# Autodesk Inventor assembly: PCB
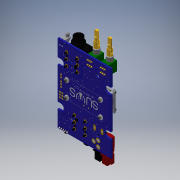
[picture p0: Inventor's stored thumbnail of the model, 180x180]
Saved by Autodesk Inventor 2016 (Build 200138000, 138)
## iProperties
Created: 2016-12-24
Part Number: PCB
Document SubType Name: Assembly
Designer: Tyler
Author: Tyler
## Documents named in this file (13)
- C:\Users\Tyler\Documents\Small Projects\Personal\morse-practice-oscillator\Mechanicial\Sounder\PCB.iam
- C:\Users\Tyler\Documents\Small Projects\Personal\morse-practice-oscillator\Mechanicial\Sounder\PCB.ipt
- C:\Users\Tyler\Documents\Small Projects\Personal\morse-practice-oscillator\Mechanicial\Sounder\Imported Components\3D+File+NRJ6HH\3D+File+NRJ6HH.ipt
- C:\Users\Tyler\Documents\Small Projects\Personal\morse-practice-oscillator\Mechanicial\Sounder\speaker.ipt
- C:\Users\Tyler\Documents\Small Projects\Personal\morse-practice-oscillator\Mechanicial\Sounder\speaker_standoff.ipt
- C:\Users\Tyler\Documents\Inventor\Content Center Files\R2016\en-US\ISO 7045  Z\ISO 7045 - M2 x 16 - 4.8 - Z - ISO.ipt
- C:\Users\Tyler\Documents\Inventor\Content Center Files\R2016\en-US\AS 1112 (2)\AS 1112 - M2  Type 5.ipt
- C:\Users\Tyler\Documents\Small Projects\Personal\morse-practice-oscillator\Mechanicial\Sounder\P082D.ipt
- C:\Users\Tyler\Documents\Small Projects\Personal\morse-practice-oscillator\Mechanicial\Sounder\Imported Components\PP 15-45 (Std)-02-08-STEP\PP 15-45 (Std)-02-08-STEP.ipt
- C:\Users\Tyler\Documents\Small Projects\Personal\morse-practice-oscillator\Mechanicial\Sounder\TE-1825232.ipt
- C:\Users\Tyler\Documents\Small Projects\Personal\morse-practice-oscillator\Mechanicial\Sounder\Multicomp-2118128.ipt
- C:\Users\Tyler\Documents\Small Projects\Personal\morse-practice-oscillator\Mechanicial\Sounder\pj-002b.ipt
- C:\Users\Tyler\Documents\Small Projects\Personal\morse-practice-oscillator\Mechanicial\Sounder\SLP3.ipt
## Components (24 placed, 12 different names)
1. PCB:1 — Flush:1, Mate:1, Mate:2, Flush:2, Mate:3, Mate:4, Insert:1, Insert:2, Insert:3, Insert:4, Insert:9, Insert:10, Insert:11, Insert:12, Mate:6, Mate:7, Flush:3, Flush:4, Mate:9, Angle:1, Mate:10, Mate:11, Mate:12, Mate:13, Mate:14, Mate:15, Mate:16, Flush:7, Flush:8, Mate:17, Flush:9, Mate:18, Mate:19, Mate:20, Mate:21, Mate:22, Flush:10, Mate:23
2. 3D+File+NRJ6HH:1 — Flush:1, Mate:1, Mate:10
3. 3D+File+NRJ6HH:2 — Mate:2, Flush:2, Mate:14
4. speaker:1 — Mate:3, Mate:4, Mate:5, Insert:5, Insert:6, Insert:7, Insert:8
5. speaker_standoff:1 — Insert:1
6. speaker_standoff:2 — Insert:2
7. speaker_standoff:3 — Insert:3, Mate:5
8. speaker_standoff:4 — Insert:4
9. ISO 7045 Z M2 x 16 - 4.8 - Z:1 — Insert:5
10. ISO 7045 Z M2 x 16 - 4.8 - Z:2 — Insert:6
11. ISO 7045 Z M2 x 16 - 4.8 - Z:3 — Insert:7
12. ISO 7045 Z M2 x 16 - 4.8 - Z:4 — Insert:8
13. AS 1112 (2) - Metric M2  Type 5:1 — Insert:9
14. AS 1112 (2) - Metric M2  Type 5:2 — Insert:10
15. AS 1112 (2) - Metric M2  Type 5:3 — Insert:11
16. AS 1112 (2) - Metric M2  Type 5:4 — Insert:12
17. P082D:1 — Mate:6, Flush:3, Mate:11
18. P082D:2 — Mate:7, Flush:4, Mate:12
19. PP 15-45 (Std)-02-08-STEP:1 — Mate:8, Flush:5, Flush:6, Mate:9, Angle:1
20. PP 15-45 (Std)-02-08-STEP:2 — Mate:8, Flush:5, Flush:6, Flush:7, Flush:8
21. TE-1825232:1 — Mate:13, Mate:15, Mate:16
22. Multicomp-2118128:1 — Mate:17, Flush:9, Mate:18
23. pj-002b:1 — Mate:19, Mate:20, Mate:21
24. SLP3:1 — Mate:22, Flush:10, Mate:23
## Relationships (46: Mate 23, Insert 12, Flush 10, Angle 1)
- Flush:1 (3.81 mm): PCB:1 ↔ 3D+File+NRJ6HH:1
- Mate:1: PCB:1 ↔ 3D+File+NRJ6HH:1
- Mate:2: PCB:1 ↔ 3D+File+NRJ6HH:2
- Flush:2 (3.81 mm): PCB:1 ↔ 3D+File+NRJ6HH:2
- Mate:3: PCB:1 ↔ speaker:1
- Mate:4: PCB:1 ↔ speaker:1
- Insert:1: PCB:1 ↔ speaker_standoff:1
- Insert:2: PCB:1 ↔ speaker_standoff:2
- Insert:3: PCB:1 ↔ speaker_standoff:3
- Insert:4: PCB:1 ↔ speaker_standoff:4
- Mate:5: speaker:1 ↔ speaker_standoff:3
- Insert:5: speaker:1 ↔ ISO 7045 Z M2 x 16 - 4.8 - Z:1
- Insert:6: speaker:1 ↔ ISO 7045 Z M2 x 16 - 4.8 - Z:2
- Insert:7: speaker:1 ↔ ISO 7045 Z M2 x 16 - 4.8 - Z:3
- Insert:8: speaker:1 ↔ ISO 7045 Z M2 x 16 - 4.8 - Z:4
- Insert:9: PCB:1 ↔ AS 1112 (2) - Metric M2  Type 5:1
- Insert:10: PCB:1 ↔ AS 1112 (2) - Metric M2  Type 5:2
- Insert:11: PCB:1 ↔ AS 1112 (2) - Metric M2  Type 5:3
- Insert:12: PCB:1 ↔ AS 1112 (2) - Metric M2  Type 5:4
- Mate:6: PCB:1 ↔ P082D:1
- Mate:7: PCB:1 ↔ P082D:2
- Flush:3: PCB:1 ↔ P082D:1
- Flush:4: PCB:1 ↔ P082D:2
- Mate:8: PP 15-45 (Std)-02-08-STEP:1 ↔ PP 15-45 (Std)-02-08-STEP:2
- Flush:5: PP 15-45 (Std)-02-08-STEP:1 ↔ PP 15-45 (Std)-02-08-STEP:2
- Flush:6: PP 15-45 (Std)-02-08-STEP:1 ↔ PP 15-45 (Std)-02-08-STEP:2
- Mate:9: PCB:1 ↔ PP 15-45 (Std)-02-08-STEP:1
- Angle:1 (180 deg): PCB:1 ↔ PP 15-45 (Std)-02-08-STEP:1
- Mate:10 (-13.97 mm): PCB:1 ↔ 3D+File+NRJ6HH:1
- Mate:11 (-34.29 mm): PCB:1 ↔ P082D:1
- Mate:12 (-48.26 mm): PCB:1 ↔ P082D:2
- Mate:13: PCB:1 ↔ TE-1825232:1
- Mate:14 (-25.4 mm): PCB:1 ↔ 3D+File+NRJ6HH:2
- Mate:15 (-6.35 mm): PCB:1 ↔ TE-1825232:1
- Mate:16 (-1.38 mm): PCB:1 ↔ TE-1825232:1
- Flush:7 (43.18 mm): PCB:1 ↔ PP 15-45 (Std)-02-08-STEP:2
- Flush:8 (69.85 mm): PCB:1 ↔ PP 15-45 (Std)-02-08-STEP:2
- Mate:17: PCB:1 ↔ Multicomp-2118128:1
- Flush:9 (-1 mm): PCB:1 ↔ Multicomp-2118128:1
- Mate:18 (-3.81 mm): PCB:1 ↔ Multicomp-2118128:1
- Mate:19: PCB:1 ↔ pj-002b:1
- Mate:20 (-86.36 mm): PCB:1 ↔ pj-002b:1
- Mate:21 (-43.18 mm): PCB:1 ↔ pj-002b:1
- Mate:22: PCB:1 ↔ SLP3:1
- Flush:10: PCB:1 ↔ SLP3:1
- Mate:23 (-3.81 mm): PCB:1 ↔ SLP3:1
